# Autodesk Inventor assembly: Screw_Sub
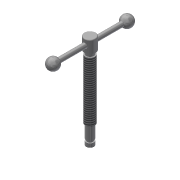
[picture p0: Inventor's stored thumbnail of the model, 180x180]
Saved by Autodesk Inventor 2022 Beta2 (Build 260130000, 130) ContinuousBuild 0
## iProperties
Created: 2006-01-18
Part Number: Screw_Sub
Document SubType Name: Assembly
Designer: PMiller
Author: PMiller
## Documents named in this file (5)
- C:\Autodesk Inventor 2021 Intro Practice Files\BOM_II\Screw_Sub.iam
- C:\Autodesk Inventor 2021 Intro Practice Files\BOM_II\Vise_Screw.ipt
- C:\Autodesk Inventor 2021 Intro Practice Files\BOM_II\Handle_Rod.ipt
- C:\Autodesk Inventor 2021 Intro Practice Files\BOM_II\Handle_Ball.ipt
- C:\Autodesk Inventor 2021 Intro Practice Files\BOM_II\Pin.ipt
## Components (6 placed, 4 different names)
1. Vise_Screw:1 — Mate:7, Mate:8
2. Handle_Rod:1 — Mate:1, Mate:2, Mate:3, Mate:4, Mate:5, Mate:6, Mate:7, Mate:8
3. Handle_Ball:1 — Mate:4, Mate:5, Mate:6, Insert:1
4. Handle_Ball:2 — Mate:1, Mate:2, Mate:3, Insert:2
5. Pin:1 — Insert:1
6. Pin:2 — Insert:2
## Relationships (10: Mate 8, Insert 2)
- Mate:1: Handle_Rod:1 ↔ Handle_Ball:2
- Mate:2: Handle_Rod:1 ↔ Handle_Ball:2
- Mate:3: Handle_Rod:1 ↔ Handle_Ball:2
- Mate:4: Handle_Rod:1 ↔ Handle_Ball:1
- Mate:5: Handle_Rod:1 ↔ Handle_Ball:1
- Mate:6: Handle_Rod:1 ↔ Handle_Ball:1
- Insert:1: Handle_Ball:1 ↔ Pin:1
- Insert:2: Handle_Ball:2 ↔ Pin:2
- Mate:7: Vise_Screw:1 ↔ Handle_Rod:1
- Mate:8: Vise_Screw:1 ↔ Handle_Rod:1
